# Autodesk Inventor assembly: Sessao8_07_04_2025_999_0001
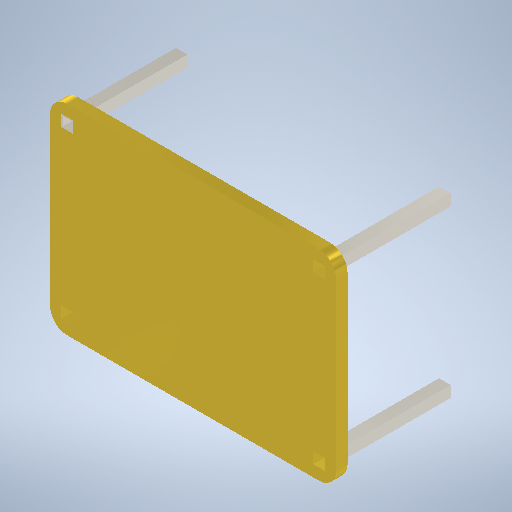
[picture p0: Inventor's stored thumbnail of the model, 512x512]
Saved by Autodesk Inventor 2025.2 (Build 292293000, 293)
## iProperties
Created: 2025-04-07
Part Number: Sessao8_07_04_2025_999_0001
Document SubType Name: Assembly
Designer: Gustavo Sousa
Author: Gustavo Sousa
## Documents named in this file (3)
- C:\Users\lucas\OneDrive\Documentos\Documentos\Gustavo\Mozangao\Robotica_Fundamentos\Inventor\Sessao8_07_04_2025\Sessao8_07_04_2025_999_0001.iam
- C:\Users\lucas\OneDrive\Documentos\Documentos\Gustavo\Mozangao\Robotica_Fundamentos\Inventor\Sessao8_07_04_2025\Sessao8_07_04_2025_0001_0001.ipt
- C:\Users\lucas\OneDrive\Documentos\Documentos\Gustavo\Mozangao\Robotica_Fundamentos\Inventor\Sessao8_07_04_2025\Sessao8_07_04_2025_0002_0001.ipt
## Components (5 placed, 2 different names)
1. Sessao8_07_04_2025_0001_0001:1 — Alinhado:1, Alinhado:2, Alinhado:3, Alinhado:4, Coincidente:2, Coincidente:3, Coincidente:4, Coincidente:5, Alinhado:10
2. Sessao8_07_04_2025_0002_0001:1 — Coincidente:5, Alinhado:6, Alinhado:8, Simetria:2
3. Sessao8_07_04_2025_0002_0001:2 — Coincidente:4, Alinhado:7, Alinhado:8
4. Sessao8_07_04_2025_0002_0001:3 — Coincidente:3, Alinhado:5, Alinhado:7, Alinhado:9, Simetria:1
5. Sessao8_07_04_2025_0002_0001:4 — Alinhado:4, Coincidente:2, Alinhado:5, Alinhado:6, Alinhado:9, Simetria:1, Simetria:2, Alinhado:10
## Relationships (16: Flush 10, Mate 4, Symmetry 2)
- Alinhado:1 [Flush]: Sessao8_07_04_2025_0001_0001:1
- Alinhado:2 [Flush]: Sessao8_07_04_2025_0001_0001:1
- Alinhado:3 [Flush]: Sessao8_07_04_2025_0001_0001:1
- Alinhado:4 [Flush] (30 mm): Sessao8_07_04_2025_0001_0001:1 ↔ Sessao8_07_04_2025_0002_0001:4
- Coincidente:2 [Mate] (-30 mm): Sessao8_07_04_2025_0001_0001:1 ↔ Sessao8_07_04_2025_0002_0001:4
- Coincidente:3 [Mate]: Sessao8_07_04_2025_0001_0001:1 ↔ Sessao8_07_04_2025_0002_0001:3
- Coincidente:4 [Mate]: Sessao8_07_04_2025_0001_0001:1 ↔ Sessao8_07_04_2025_0002_0001:2
- Coincidente:5 [Mate]: Sessao8_07_04_2025_0001_0001:1 ↔ Sessao8_07_04_2025_0002_0001:1
- Alinhado:5 [Flush]: Sessao8_07_04_2025_0002_0001:3 ↔ Sessao8_07_04_2025_0002_0001:4
- Alinhado:6 [Flush]: Sessao8_07_04_2025_0002_0001:1 ↔ Sessao8_07_04_2025_0002_0001:4
- Alinhado:7 [Flush]: Sessao8_07_04_2025_0002_0001:2 ↔ Sessao8_07_04_2025_0002_0001:3
- Alinhado:8 [Flush]: Sessao8_07_04_2025_0002_0001:1 ↔ Sessao8_07_04_2025_0002_0001:2
- Alinhado:9 [Flush]: Sessao8_07_04_2025_0002_0001:3 ↔ Sessao8_07_04_2025_0002_0001:4
- Simetria:1 [Symmetry]: Sessao8_07_04_2025_0002_0001:3 ↔ Sessao8_07_04_2025_0002_0001:4
- Simetria:2 [Symmetry]: Sessao8_07_04_2025_0002_0001:1 ↔ Sessao8_07_04_2025_0002_0001:4
- Alinhado:10 [Flush]: Sessao8_07_04_2025_0001_0001:1 ↔ Sessao8_07_04_2025_0002_0001:4
